# Autodesk Inventor assembly: pat
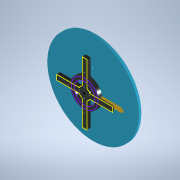
[picture p0: Inventor's stored thumbnail of the model, 180x180]
Saved by Autodesk Inventor 2022 (Build 260153000, 153)
## iProperties
Created: 2022-02-27
Part Number: pat
Document SubType Name: Assembly
Designer: Oana
Author: Oana
## Documents named in this file (6)
- D:\salvari\aplicatii-proiecte\infoeducatia 2022\cad final sper\Scanner3D\infoeducatia 2022\proiectare\pat_scanare\pat.iam
- D:\salvari\aplicatii-proiecte\infoeducatia 2022\cad final sper\Scanner3D\infoeducatia 2022\proiectare\pat_scanare\pat.ipt
- D:\salvari\aplicatii-proiecte\infoeducatia 2022\cad final sper\Scanner3D\infoeducatia 2022\proiectare\pat_scanare\suport + senzor.iam
- D:\salvari\aplicatii-proiecte\infoeducatia 2022\cad final sper\Scanner3D\infoeducatia 2022\proiectare\piese\39172_txm-axle hub with set screw (1).ipt
- D:\salvari\aplicatii-proiecte\infoeducatia 2022\cad final sper\Scanner3D\infoeducatia 2022\proiectare\pat_scanare\tija.ipt
- C:\Users\Miss Oana\Desktop\Part1.ipt
## Components (5 placed, 5 different names)
1. pat:1 — Rotational:1, Rotational:3
2. suport + senzor:1 [sub-assembly] — Rotational:1, Rotational:2, Rotational:4
3. 39172_txm-axle hub with set screw (1):1 — Rotational:2, Rigid:4
4. tija:1 — Rigid:4
5. Part1:1 — Rotational:3, Rotational:4
## Relationships (5: RevoluteJoint 4, WeldJoint 1)
- Rotational:1 [RevoluteJoint]: pat:1 ↔ suport + senzor:1
- Rotational:2 [RevoluteJoint]: suport + senzor:1 ↔ 39172_txm-axle hub with set screw (1):1
- Rigid:4 [WeldJoint]: 39172_txm-axle hub with set screw (1):1 ↔ tija:1
- Rotational:3 [RevoluteJoint]: pat:1 ↔ Part1:1
- Rotational:4 [RevoluteJoint]: suport + senzor:1 ↔ Part1:1
